# Autodesk Inventor assembly: Gripper
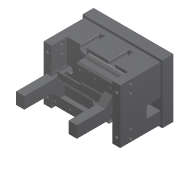
[picture p0: Inventor's stored thumbnail of the model, 180x180]
Saved by Autodesk Inventor 2017 (Build 210142000, 142)
## iProperties
Created: 2018-10-23
Part Number: Gripper
Document SubType Name: Assembly
Designer: Dell
Author: Dell
## Documents named in this file (9)
- C:\Users\Dell\Documents\GitHub\tr2\Gripper\Gripper.iam
- C:\Users\Dell\Documents\GitHub\tr2\Gripper\AX-12A.ipt
- C:\Users\Dell\Documents\GitHub\tr2\Gripper\Gripper\Design Accelerator\Spur Gears1.iam
- C:\Users\Dell\Documents\GitHub\tr2\Gripper\GA04.ipt
- C:\Users\Dell\Documents\GitHub\tr2\Gripper\GA01b.ipt
- C:\Users\Dell\Documents\GitHub\tr2\Gripper\GA05.ipt
- C:\Users\Dell\Documents\GitHub\tr2\Gripper\GA06.ipt
- C:\Users\Dell\Documents\GitHub\tr2\Gripper\GA07.ipt
- C:\Users\Dell\Documents\GitHub\tr2\Gripper\GA08.ipt
## Components (9 placed, 8 different names)
1. GA01b:1 — Mate:24, Mate:25, Mate:26, Mate:28, Mate:29, Mate:30, Mate:31, Mate:42, Mate:43, Mate:44, Mate:48, Mate:49, Mate:50, Mate:51, Mate:52, Mate:53, Mate:54, Mate:55, Mate:56, Mate:57
2. AX-12A:2 — Mate:24, Mate:25, Mate:26, Mate:58
3. GA04:3 — Mate:28, Rotation/Translation:3, Mate:33, Mate:34, Mate:38, Mate:44
4. GA04:4 — Mate:29, Mate:30, Rotation/Translation:4, Mate:45, Mate:46, Mate:47
5. Spur Gears:2 [sub-assembly] — Mate:31, Rotation/Translation:3, Rotation/Translation:4, Mate:58
6. GA05:1 — Mate:33, Mate:34, Mate:38, Mate:53
7. GA06:1 — Mate:42, Mate:43, Mate:51
8. GA07:1 — Mate:45, Mate:46, Mate:47, Mate:54
9. GA08:1 — Mate:55, Mate:56, Mate:57
## Relationships (29: Mate 27, RelateRotateTranslate 2)
- Mate:24: GA01b:1 ↔ AX-12A:2
- Mate:25: GA01b:1 ↔ AX-12A:2
- Mate:26: GA01b:1 ↔ AX-12A:2
- Mate:28: GA01b:1 ↔ GA04:3
- Mate:29: GA01b:1 ↔ GA04:4
- Mate:30: GA01b:1 ↔ GA04:4
- Mate:31: GA01b:1 ↔ Spur Gears:2
- Rotation/Translation:3 [RelateRotateTranslate] (131 mm): GA04:3 ↔ Spur Gears:2
- Rotation/Translation:4 [RelateRotateTranslate] (131 mm): GA04:4 ↔ Spur Gears:2
- Mate:33: GA04:3 ↔ GA05:1
- Mate:34: GA04:3 ↔ GA05:1
- Mate:38: GA04:3 ↔ GA05:1
- Mate:42: GA01b:1 ↔ GA06:1
- Mate:43: GA01b:1 ↔ GA06:1
- Mate:44: GA01b:1 ↔ GA04:3
- Mate:45: GA04:4 ↔ GA07:1
- Mate:46: GA04:4 ↔ GA07:1
- Mate:47: GA04:4 ↔ GA07:1
- Mate:48: GA01b:1
- Mate:49: GA01b:1
- Mate:50: GA01b:1
- Mate:51: GA01b:1 ↔ GA06:1
- Mate:52: GA01b:1
- Mate:53: GA01b:1 ↔ GA05:1
- Mate:54: GA01b:1 ↔ GA07:1
- Mate:55: GA01b:1 ↔ GA08:1
- Mate:56: GA01b:1 ↔ GA08:1
- Mate:57: GA01b:1 ↔ GA08:1
- Mate:58: AX-12A:2 ↔ Spur Gears:2
